# Autodesk Inventor assembly: FRC Arena 2013 (TEST VERSION) - top rung - 26x28 arpan version
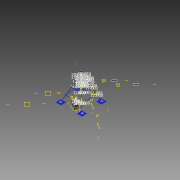
[picture p0: Inventor's stored thumbnail of the model, 180x180]
Saved by Autodesk Inventor 2013 (Build 170138000, 138)
## iProperties
Created: 2013-01-07
Part Number: FRC Arena 2013 (TEST VERSION) - top rung - 26x28 arpan version
Document SubType Name: Assembly
Designer: Phillip
Author: Phillip
## Documents named in this file (7)
- C:\Users\Arpan\Documents\GitHub\frc2013CAD\FIRST Arena 2013\FRC Arena 2013 (TEST VERSION) - top rung - 26x28 arpan version.iam
- C:\Users\Arpan\Documents\GitHub\frc2013CAD\FIRST Arena 2013\Arena\Arena Base.ipt
- C:\Users\Arpan\Documents\GitHub\frc2013CAD\FIRST Arena 2013\Pyramid\GE-13017.iam
- C:\Users\Arpan\Documents\GitHub\frc2013CAD\FIRST Arena 2013\Playing Configuration Constraint.ipt
- C:\Users\Arpan\Documents\GitHub\frc2013CAD\Cimber actual\Part4.ipt
- C:\Users\Arpan\Documents\GitHub\frc2013CAD\Cimber actual\Part5.ipt
- C:\Users\Arpan\Documents\GitHub\frc2013CAD\arpans version robot.iam
## Components (6 placed, 6 different names)
1. Arena Base:1 — Mate:2, Angle:1, Mate:3, Angle:2, Flush:3
2. GE-13017:1 [sub-assembly] — Angle:3
3. Playing Configuration Constraint:1
4. Part4:1
5. Part5:1
6. arpans version robot:1 [sub-assembly] — Angle:3
## Relationships (8: Angle 3, Flush 3, Mate 2)
- Mate:2: Arena Base:1
- Angle:1 (0 deg): Arena Base:1
- Flush:1 (2743.2 mm)
- Mate:3: Arena Base:1
- Angle:2 (0 deg): Arena Base:1
- Flush:2 (-2743.2 mm)
- Flush:3: Arena Base:1
- Angle:3 (0 deg): GE-13017:1 ↔ arpans version robot:1
